# Autodesk Inventor assembly: 8100_Tx_Filter_Layout_v1
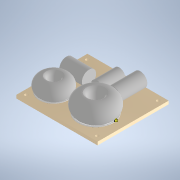
[picture p0: Inventor's stored thumbnail of the model, 180x180]
Saved by Autodesk Inventor 2021 (Build 250183000, 183)
## iProperties
Created: 2021-03-01
Part Number: 8100_Tx_Filter_Layout_v1
Document SubType Name: Assembly
Designer: Barksdale
Author: Barksdale
## Documents named in this file (9)
- C:\Users\Barksdale\Dropbox (MIT)\MPI Group Folder\MPS\Inventor_Parts\MPSV2\Tx Filter\8100_Tx_Filter_Layout_v1.iam
- C:\Users\Barksdale\Dropbox (MIT)\MPI Group Folder\MPS\Inventor_Parts\MPSV2\Tx Filter\8010_2uF_Tx_Capacitor_v1.ipt
- C:\Users\Barksdale\Dropbox (MIT)\MPI Group Folder\MPS\Inventor_Parts\MPSV2\Tx Filter\8011_1uF_Tx_Capacitor_v1.ipt
- C:\Users\Barksdale\Dropbox (MIT)\MPI Group Folder\MPS\Inventor_Parts\MPSV2\Tx Filter\8012_560nF_Tx_Capacitor_v1.ipt
- C:\Users\Barksdale\Dropbox (MIT)\MPI Group Folder\MPS\Inventor_Parts\MPSV2\Tx Filter\8000_132uH_DCore_2layer_Tx_Filter_MPSv2_v1.ipt
- C:\Users\Barksdale\Dropbox (MIT)\MPI Group Folder\MPS\Inventor_Parts\MPSV2\Tx Filter\8001_250uH_DCore_2layer_Tx_Filter_MPSv2_v1.ipt
- C:\Users\Barksdale\Dropbox (MIT)\MPI Group Folder\MPS\Inventor_Parts\MPSV2\Tx Filter\8020_Base_Tx_Filter_v1.ipt
- C:\Users\Barksdale\Dropbox (MIT)\MPI Group Folder\MPS\Inventor_Parts\MPSV2\Tx Filter\8003_base_250uH_DCore_2layer_Tx_Filter_MPSv2_v3.ipt
- C:\Users\Barksdale\Dropbox (MIT)\MPI Group Folder\MPS\Inventor_Parts\MPSV2\Tx Filter\8002_base_132uH_DCore_2layer_Tx_Filter_MPSv2_v1.ipt
## Components (8 placed, 8 different names)
1. 8010_2uF_Tx_Capacitor_v1:1 — Tangent:3
2. 8011_1uF_Tx_Capacitor_v1:1 — Tangent:2
3. 8012_560nF_Tx_Capacitor_v1:1 — Tangent:1
4. 8000_132uH_DCore_2layer_Tx_Filter_MPSv2_v1:1 — Mate:4
5. 8001_250uH_DCore_2layer_Tx_Filter_MPSv2_v1:1 — Mate:3
6. 8020_Base_Tx_Filter_v1:1 — Mate:1, Mate:2, Tangent:1, Tangent:2, Tangent:3
7. 8003_base_250uH_DCore_2layer_Tx_Filter_MPSv2_v3:1 — Mate:2, Mate:3
8. 8002_base_132uH_DCore_2layer_Tx_Filter_MPSv2_v1:1 — Mate:1, Mate:4
## Relationships (7: Mate 4, Tangent 3)
- Mate:1: 8020_Base_Tx_Filter_v1:1 ↔ 8002_base_132uH_DCore_2layer_Tx_Filter_MPSv2_v1:1
- Mate:2: 8020_Base_Tx_Filter_v1:1 ↔ 8003_base_250uH_DCore_2layer_Tx_Filter_MPSv2_v3:1
- Mate:3: 8001_250uH_DCore_2layer_Tx_Filter_MPSv2_v1:1 ↔ 8003_base_250uH_DCore_2layer_Tx_Filter_MPSv2_v3:1
- Mate:4: 8000_132uH_DCore_2layer_Tx_Filter_MPSv2_v1:1 ↔ 8002_base_132uH_DCore_2layer_Tx_Filter_MPSv2_v1:1
- Tangent:1: 8012_560nF_Tx_Capacitor_v1:1 ↔ 8020_Base_Tx_Filter_v1:1
- Tangent:2: 8011_1uF_Tx_Capacitor_v1:1 ↔ 8020_Base_Tx_Filter_v1:1
- Tangent:3: 8010_2uF_Tx_Capacitor_v1:1 ↔ 8020_Base_Tx_Filter_v1:1
